# Autodesk Inventor assembly: Camera & Angle
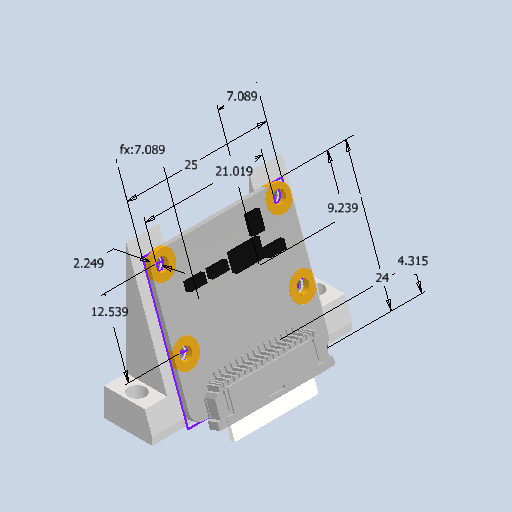
[picture p0: Inventor's stored thumbnail of the model, 512x512]
Saved by Autodesk Inventor 2022 (Build 260153000, 153)
## iProperties
Created: 2023-03-10
Part Number: Camera & Angle
Document SubType Name: Assembly
Designer: zarek
Author: zarek
## Documents named in this file (3)
- C:\Users\zarek\OneDrive\Desktop\Random New Stuff\SPB\Camera & Angle.iam
- C:\Users\zarek\OneDrive\Desktop\Random New Stuff\SPB\Camera Angle.ipt
- C:\Users\zarek\OneDrive\Desktop\Random New Stuff\SPB\GrabCad Parts\Camera Moudule 3 v8.iam
## Components (2 placed, 2 different names)
1. Camera Angle:1 — Rigid:1
2. Camera Moudule 3 v8:1 [sub-assembly] — Rigid:1
## Relationships (1: WeldJoint 1)
- Rigid:1 [WeldJoint] (1 mm): Camera Angle:1 ↔ Camera Moudule 3 v8:1
